# Autodesk Inventor assembly: Seringa
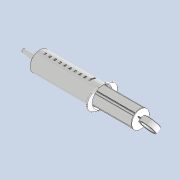
[picture p0: Inventor's stored thumbnail of the model, 180x180]
Saved by Autodesk Inventor 2020 (Build 240168000, 168)
## iProperties
Created: 2021-05-19
Part Number: Seringa
Document SubType Name: Assembly
Designer: Iulian Bors
Author: Iulian Bors
## Documents named in this file (4)
- Z:\I.A.B\Proiecte\0008 I.A.B 3D 2.1 Imprimanta aracet Metal\30 Injectomat\syringe-100ml-1.snapshot.1\Seringa.iam
- Z:\I.A.B\Proiecte\0008 I.A.B 3D 2.1 Imprimanta aracet Metal\30 Injectomat\syringe-100ml-1.snapshot.1\Cauciuc.ipt
- Z:\I.A.B\Proiecte\0008 I.A.B 3D 2.1 Imprimanta aracet Metal\30 Injectomat\syringe-100ml-1.snapshot.1\Corp.ipt
- Z:\I.A.B\Proiecte\0008 I.A.B 3D 2.1 Imprimanta aracet Metal\30 Injectomat\syringe-100ml-1.snapshot.1\Syringe_100ml.ipt
## Components (3 placed, 3 different names)
1. Cauciuc:1 — Insert:1, Mate:1
2. Corp:1 — Mate:1
3. Syringe_100ml:1 — Insert:1
## Relationships (2: Insert 1, Mate 1)
- Insert:1: Cauciuc:1 ↔ Syringe_100ml:1
- Mate:1: Cauciuc:1 ↔ Corp:1
